# Autodesk Inventor assembly: Weapon Assembly
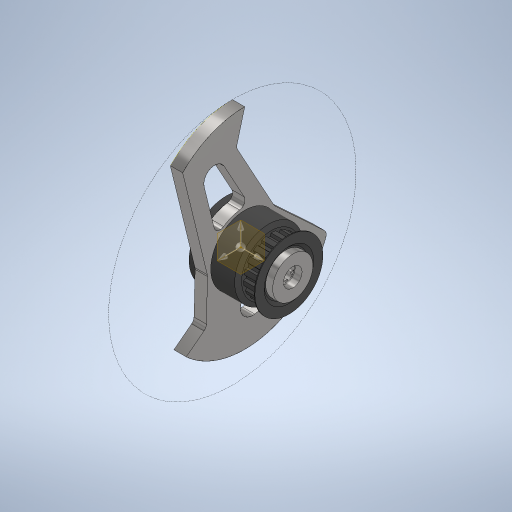
[picture p0: Inventor's stored thumbnail of the model, 512x512]
Saved by Autodesk Inventor 2023.4 (Build 274418000, 418)
## iProperties
Created: 2023-11-14
Part Number: Weapon Assembly
Document SubType Name: Assembly
Designer: Nathan Cai
Mass: 234.695 g
Surface Area: 238.219 cm^2
Volume: 40.7425 cm^3
Author: Nathan Cai
## Documents named in this file (6)
- E:\Documents\Inventor\Chort V2.1\Weapon Assembly.iam
- E:\Documents\Inventor\Chort V2.1\Blade.ipt
- E:\Documents\Inventor\Chort V2.1\XL Pulley 18T .25in Wd - ++.ipt
- E:\Documents\Inventor\Chort V2.1\Needle Bearings.ipt
- E:\Documents\Inventor\Chort V2.1\5905K497_Needle-Roller Bearing (1).ipt
- E:\Documents\Inventor\Chort V2.1\Spacer 3-8x .125.ipt
## Components (7 placed, 5 different names)
1. Blade:1 — Mate:1, Mate:2, Mate:3, Mate:5, Flush:2, Mate:7, Mate:8, Mate:10
2. XL Pulley 18T .25in Wd - ++:1 — Mate:1, Mate:2, Mate:3, Mate:4, Mate:13, Flush:3
3. Needle Bearings:1 — Mate:7, Mate:13
4. Needle Bearings:2 — Mate:11, Mate:12
5. 5905K497_Needle-Roller Bearing (1):1 — Mate:4, Flush:3
6. 5905K497_Needle-Roller Bearing (1):2 — Mate:5, Flush:2, Mate:9
7. Spacer 3-8x .125:1 — Mate:8, Mate:9, Mate:10, Mate:11, Mate:12
## Relationships (14: Mate 12, Flush 2)
- Mate:1: Blade:1 ↔ XL Pulley 18T .25in Wd - ++:1
- Mate:2: Blade:1 ↔ XL Pulley 18T .25in Wd - ++:1
- Mate:3: Blade:1 ↔ XL Pulley 18T .25in Wd - ++:1
- Mate:4: XL Pulley 18T .25in Wd - ++:1 ↔ 5905K497_Needle-Roller Bearing (1):1
- Mate:5: Blade:1 ↔ 5905K497_Needle-Roller Bearing (1):2
- Flush:2 (-1.5875 mm): Blade:1 ↔ 5905K497_Needle-Roller Bearing (1):2
- Mate:7: Blade:1 ↔ Needle Bearings:1
- Mate:8: Blade:1 ↔ Spacer 3-8x .125:1
- Mate:9: 5905K497_Needle-Roller Bearing (1):2 ↔ Spacer 3-8x .125:1
- Mate:10: Blade:1 ↔ Spacer 3-8x .125:1
- Mate:11: Needle Bearings:2 ↔ Spacer 3-8x .125:1
- Mate:12: Needle Bearings:2 ↔ Spacer 3-8x .125:1
- Mate:13: XL Pulley 18T .25in Wd - ++:1 ↔ Needle Bearings:1
- Flush:3: XL Pulley 18T .25in Wd - ++:1 ↔ 5905K497_Needle-Roller Bearing (1):1
